# Autodesk Inventor assembly: SolarAssembly
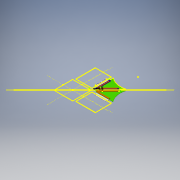
[picture p0: Inventor's stored thumbnail of the model, 180x180]
Saved by Autodesk Inventor 2016 (Build 200138000, 138)
## iProperties
Created: 2015-06-07
Part Number: SolarAssembly
Document SubType Name: Assembly
Designer: Erin
Author: Erin
## Documents named in this file (4)
- C:\Users\Erin\Desktop\RDAS v0.2\SolarAssembly.iam
- C:\Users\Erin\Desktop\RDAS v0.2\SolarFolds_Sketch-Flex.ipt
- C:\Users\Erin\Desktop\RDAS v0.2\SolarFolds_Sketch-Panel-Mirror.ipt
- C:\Users\Erin\Desktop\RDAS v0.2\SolarFolds_Sketch-Clamp.ipt
## Components (4 placed, 3 different names)
1. SolarFolds_Sketch-Flex:1 — Insert:1, Insert:2
2. SolarFolds_Sketch-Panel-Mirror:1 — Insert:1
3. SolarFolds_Sketch-Panel-Mirror:2 — Insert:2
4. SolarFolds_Sketch-Clamp:1
## Relationships (2: Insert 2)
- Insert:1: SolarFolds_Sketch-Flex:1 ↔ SolarFolds_Sketch-Panel-Mirror:1
- Insert:2: SolarFolds_Sketch-Flex:1 ↔ SolarFolds_Sketch-Panel-Mirror:2
